# Autodesk Inventor assembly: Assembly1
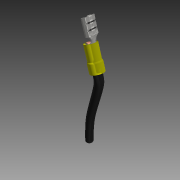
[picture p0: Inventor's stored thumbnail of the model, 180x180]
Saved by Autodesk Inventor 2014 (Build 180170000, 170)
## iProperties
Created: 2013-07-21
Part Number: Assembly1
Document SubType Name: Assembly
Designer: Saville
Mass: 1.02747 g
Surface Area: 17.3563 cm^2
Volume: 1.02747 cm^3
Density: 1 g/cm^3
Author: Saville
## Documents named in this file (3)
- C:\electrical nuts\terminal\12-10 female spade yellow\Assembly1.iam
- C:\electrical nuts\terminal\12-10 female spade yellow\WIRE.ipt
- C:\electrical nuts\terminal\12-10 female spade yellow\12-10 female flat spade yellow.ipt
## Components (2 placed, 2 different names)
1. WIRE:1 — Mate:1, Mate:2, Flush:1
2. 12-10 female flat spade yellow:1 — Mate:2, Flush:1
## Relationships (3: Mate 2, Flush 1)
- Mate:1: WIRE:1
- Mate:2: WIRE:1 ↔ 12-10 female flat spade yellow:1
- Flush:1 (-0.381 mm): WIRE:1 ↔ 12-10 female flat spade yellow:1
